# Autodesk Inventor assembly: DriverStation-ver2-1111-2021
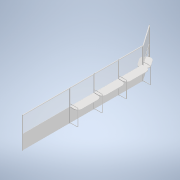
[picture p0: Inventor's stored thumbnail of the model, 180x180]
Saved by Autodesk Inventor 2021 (Build 250183000, 183)
## iProperties
Created: 2021-03-02
Part Number: DriverStation-ver2-1111-2021
Document SubType Name: Assembly
Designer: CMurray
Author: CMurray
## Documents named in this file (14)
- F:\PHRC CADD 2021\2021 Game Design Challenge\Player Station\Assemblies\DriverStation-ver2-1111-2021.iam
- F:\PHRC CADD 2021\2021 Game Design Challenge\Player Station\Parts\StationBase-ver1-1111-2021.ipt
- F:\PHRC CADD 2021\2021 Game Design Challenge\Player Station\Parts\StationDivider-ver1-1111-2021.iam
- F:\PHRC CADD 2021\2021 Game Design Challenge\Player Station\Parts\HPStationBase-ver1-1111-2021.ipt
- F:\PHRC CADD 2021\2021 Game Design Challenge\Player Station\Parts\StationDividerNoArm-ver1-1111-2021.iam
- F:\PHRC CADD 2021\2021 Game Design Challenge\Player Station\Parts\PSHalfWall-ver2-1111-2021.ipt
- F:\PHRC CADD 2021\2021 Game Design Challenge\Player Station\Parts\StationWindow-ver1-1111-2021.ipt
- F:\PHRC CADD 2021\2021 Game Design Challenge\Player Station\Parts\TopBar-ver1-1111-2021.ipt
- F:\PHRC CADD 2021\2021 Game Design Challenge\Player Station\Parts\TopBar-ver2-1111-2021.ipt
- F:\PHRC CADD 2021\2021 Game Design Challenge\Player Station\Parts\StationWindow-ver2-1111-2021.ipt
- F:\PHRC CADD 2021\2021 Game Design Challenge\Player Station\Parts\TopBar-ver3-1111-2021.ipt
- F:\PHRC CADD 2021\2021 Game Design Challenge\Player Station\Parts\StationWindow-ver3-1111-2021.ipt
- F:\PHRC CADD 2021\2021 Game Design Challenge\Player Station\Parts\Shelf-ver1-1111-2021.ipt
- F:\PHRC CADD 2021\2021 Game Design Challenge\Player Station\Parts\Shelf-ver2-1111-2021.ipt
## Components (26 placed, 13 different names)
1. StationBase-ver1-1111-2021:1 — Mate:1, Flush:1, Flush:2, Flush:3, Mate:2, Flush:4, Flush:7, Flush:8, Flush:11, Flush:12, Mate:21, Flush:34, Flush:40, Mate:30
2. StationDivider-ver1-1111-2021:1 [sub-assembly] — Mate:1, Flush:1, Flush:2, Mate:6, Mate:14, Flush:23, Flush:24, Mate:24, Mate:31
3. StationDivider-ver1-1111-2021:2 [sub-assembly] — Flush:3, Mate:2, Flush:4, Mate:4, Angle:2, Mate:15, Flush:25, Flush:26, Mate:22, Mate:33
4. StationBase-ver1-1111-2021:2 — Mate:4, Flush:7, Flush:8, Mate:9, Flush:16, Flush:17, Angle:3, Mate:19, Flush:33, Flush:41, Mate:32
5. StationBase-ver1-1111-2021:3 — Flush:11, Flush:12, Mate:6, Flush:19, Flush:20, Mate:23, Flush:35, Mate:28, Mate:29, Flush:39
6. StationDivider-ver1-1111-2021:4 [sub-assembly] — Mate:12, Flush:37, Mate:27
7. StationDivider-ver1-1111-2021:6 [sub-assembly] — Mate:9, Flush:16, Angle:2, Mate:10, Angle:4, Mate:16, Flush:27, Flush:28, Mate:20
8. HPStationBase-ver1-1111-2021:1 — Mate:10, Flush:17, Angle:3, Mate:11, Flush:18, Flush:29, Mate:17, Flush:30, Mate:34, Mate:35, Flush:42, Mate:36, Mate:37
9. StationDividerNoArm-ver1-1111-2021:1 [sub-assembly] — Mate:11, Angle:4, Flush:18
10. PSHalfWall-ver2-1111-2021:1 — Flush:19, Flush:20, Mate:12, Mate:13, Flush:21, Flush:22, Flush:36, Flush:38, Mate:26
11. StationDividerNoArm-ver1-1111-2021:2 [sub-assembly] — Mate:13, Flush:21, Flush:22, Mate:25
12. TopBar-ver1-1111-2021:1 — Mate:14, Flush:23, Flush:24
13. TopBar-ver1-1111-2021:2 — Mate:15, Flush:25, Flush:26
14. TopBar-ver1-1111-2021:3 — Mate:16, Flush:27, Flush:28
15. StationWindow-ver2-1111-2021:1 — Flush:29, Mate:17, Flush:30, Mate:18, Flush:31, Flush:32
16. TopBar-ver2-1111-2021:2 — Mate:18, Flush:31, Flush:32
17. StationWindow-ver1-1111-2021:1 — Mate:19, Flush:33, Mate:20
18. StationWindow-ver1-1111-2021:2 — Mate:21, Flush:34, Mate:22
19. StationWindow-ver1-1111-2021:3 — Mate:23, Flush:35, Mate:24
20. TopBar-ver3-1111-2021:1 — Mate:25, Flush:36, Flush:37
21. StationWindow-ver3-1111-2021:1 — Flush:38, Mate:26, Mate:27
22. Shelf-ver1-1111-2021:1 — Mate:28, Mate:29, Flush:39
23. Shelf-ver1-1111-2021:2 — Flush:40, Mate:30, Mate:31
24. Shelf-ver1-1111-2021:3 — Flush:41, Mate:32, Mate:33
25. Shelf-ver2-1111-2021:1 — Mate:34, Mate:35, Flush:42, Flush:43
26. Shelf-ver2-1111-2021:2 — Mate:36, Flush:43, Mate:37
## Relationships (75: Flush 38, Mate 34, Angle 3)
- Mate:1: StationBase-ver1-1111-2021:1 ↔ StationDivider-ver1-1111-2021:1
- Flush:1: StationBase-ver1-1111-2021:1 ↔ StationDivider-ver1-1111-2021:1
- Flush:2: StationBase-ver1-1111-2021:1 ↔ StationDivider-ver1-1111-2021:1
- Flush:3: StationBase-ver1-1111-2021:1 ↔ StationDivider-ver1-1111-2021:2
- Mate:2: StationBase-ver1-1111-2021:1 ↔ StationDivider-ver1-1111-2021:2
- Flush:4: StationBase-ver1-1111-2021:1 ↔ StationDivider-ver1-1111-2021:2
- Mate:4: StationDivider-ver1-1111-2021:2 ↔ StationBase-ver1-1111-2021:2
- Flush:7: StationBase-ver1-1111-2021:1 ↔ StationBase-ver1-1111-2021:2
- Flush:8: StationBase-ver1-1111-2021:1 ↔ StationBase-ver1-1111-2021:2
- [Mate]: StationBase-ver1-1111-2021:3 ↔ StationDivider-ver1-1111-2021:4
- [Flush]: StationBase-ver1-1111-2021:3 ↔ StationDivider-ver1-1111-2021:4
- [Flush]: StationBase-ver1-1111-2021:3 ↔ StationDivider-ver1-1111-2021:4
- Flush:11: StationBase-ver1-1111-2021:1 ↔ StationBase-ver1-1111-2021:3
- Flush:12: StationBase-ver1-1111-2021:1 ↔ StationBase-ver1-1111-2021:3
- Mate:6: StationDivider-ver1-1111-2021:1 ↔ StationBase-ver1-1111-2021:3
- Mate:9: StationBase-ver1-1111-2021:2 ↔ StationDivider-ver1-1111-2021:6
- Flush:16: StationBase-ver1-1111-2021:2 ↔ StationDivider-ver1-1111-2021:6
- Angle:2 (0 deg): StationDivider-ver1-1111-2021:2 ↔ StationDivider-ver1-1111-2021:6
- Mate:10: StationDivider-ver1-1111-2021:6 ↔ HPStationBase-ver1-1111-2021:1
- Flush:17: StationBase-ver1-1111-2021:2 ↔ HPStationBase-ver1-1111-2021:1
- Angle:3 (35 deg): StationBase-ver1-1111-2021:2 ↔ HPStationBase-ver1-1111-2021:1
- Mate:11: HPStationBase-ver1-1111-2021:1 ↔ StationDividerNoArm-ver1-1111-2021:1
- Angle:4 (0 deg): StationDivider-ver1-1111-2021:6 ↔ StationDividerNoArm-ver1-1111-2021:1
- Flush:18: HPStationBase-ver1-1111-2021:1 ↔ StationDividerNoArm-ver1-1111-2021:1
- Flush:19: StationBase-ver1-1111-2021:3 ↔ PSHalfWall-ver2-1111-2021:1
- Flush:20: StationBase-ver1-1111-2021:3 ↔ PSHalfWall-ver2-1111-2021:1
- Mate:12: StationDivider-ver1-1111-2021:4 ↔ PSHalfWall-ver2-1111-2021:1
- Mate:13: PSHalfWall-ver2-1111-2021:1 ↔ StationDividerNoArm-ver1-1111-2021:2
- Flush:21: PSHalfWall-ver2-1111-2021:1 ↔ StationDividerNoArm-ver1-1111-2021:2
- Flush:22: PSHalfWall-ver2-1111-2021:1 ↔ StationDividerNoArm-ver1-1111-2021:2
- Mate:14: StationDivider-ver1-1111-2021:1 ↔ TopBar-ver1-1111-2021:1
- Flush:23: StationDivider-ver1-1111-2021:1 ↔ TopBar-ver1-1111-2021:1
- Flush:24: StationDivider-ver1-1111-2021:1 ↔ TopBar-ver1-1111-2021:1
- Mate:15: StationDivider-ver1-1111-2021:2 ↔ TopBar-ver1-1111-2021:2
- Flush:25: StationDivider-ver1-1111-2021:2 ↔ TopBar-ver1-1111-2021:2
- Flush:26: StationDivider-ver1-1111-2021:2 ↔ TopBar-ver1-1111-2021:2
- Mate:16: StationDivider-ver1-1111-2021:6 ↔ TopBar-ver1-1111-2021:3
- Flush:27: StationDivider-ver1-1111-2021:6 ↔ TopBar-ver1-1111-2021:3
- Flush:28: StationDivider-ver1-1111-2021:6 ↔ TopBar-ver1-1111-2021:3
- Flush:29: HPStationBase-ver1-1111-2021:1 ↔ StationWindow-ver2-1111-2021:1
- Mate:17: HPStationBase-ver1-1111-2021:1 ↔ StationWindow-ver2-1111-2021:1
- Flush:30: HPStationBase-ver1-1111-2021:1 ↔ StationWindow-ver2-1111-2021:1
- Mate:18: StationWindow-ver2-1111-2021:1 ↔ TopBar-ver2-1111-2021:2
- Flush:31: StationWindow-ver2-1111-2021:1 ↔ TopBar-ver2-1111-2021:2
- Flush:32: StationWindow-ver2-1111-2021:1 ↔ TopBar-ver2-1111-2021:2
- Mate:19: StationBase-ver1-1111-2021:2 ↔ StationWindow-ver1-1111-2021:1
- Flush:33: StationBase-ver1-1111-2021:2 ↔ StationWindow-ver1-1111-2021:1
- Mate:20: StationDivider-ver1-1111-2021:6 ↔ StationWindow-ver1-1111-2021:1
- Mate:21: StationBase-ver1-1111-2021:1 ↔ StationWindow-ver1-1111-2021:2
- Flush:34: StationBase-ver1-1111-2021:1 ↔ StationWindow-ver1-1111-2021:2
- Mate:22: StationDivider-ver1-1111-2021:2 ↔ StationWindow-ver1-1111-2021:2
- Mate:23: StationBase-ver1-1111-2021:3 ↔ StationWindow-ver1-1111-2021:3
- Flush:35: StationBase-ver1-1111-2021:3 ↔ StationWindow-ver1-1111-2021:3
- Mate:24: StationDivider-ver1-1111-2021:1 ↔ StationWindow-ver1-1111-2021:3
- Mate:25: StationDividerNoArm-ver1-1111-2021:2 ↔ TopBar-ver3-1111-2021:1
- Flush:36: PSHalfWall-ver2-1111-2021:1 ↔ TopBar-ver3-1111-2021:1
- Flush:37: StationDivider-ver1-1111-2021:4 ↔ TopBar-ver3-1111-2021:1
- Flush:38: PSHalfWall-ver2-1111-2021:1 ↔ StationWindow-ver3-1111-2021:1
- Mate:26: PSHalfWall-ver2-1111-2021:1 ↔ StationWindow-ver3-1111-2021:1
- Mate:27: StationDivider-ver1-1111-2021:4 ↔ StationWindow-ver3-1111-2021:1
- Mate:28: StationBase-ver1-1111-2021:3 ↔ Shelf-ver1-1111-2021:1
- Mate:29: StationBase-ver1-1111-2021:3 ↔ Shelf-ver1-1111-2021:1
- Flush:39: StationBase-ver1-1111-2021:3 ↔ Shelf-ver1-1111-2021:1
- Flush:40: StationBase-ver1-1111-2021:1 ↔ Shelf-ver1-1111-2021:2
- Mate:30: StationBase-ver1-1111-2021:1 ↔ Shelf-ver1-1111-2021:2
- Mate:31: StationDivider-ver1-1111-2021:1 ↔ Shelf-ver1-1111-2021:2
- Flush:41: StationBase-ver1-1111-2021:2 ↔ Shelf-ver1-1111-2021:3
- Mate:32: StationBase-ver1-1111-2021:2 ↔ Shelf-ver1-1111-2021:3
- Mate:33: StationDivider-ver1-1111-2021:2 ↔ Shelf-ver1-1111-2021:3
- Mate:34: HPStationBase-ver1-1111-2021:1 ↔ Shelf-ver2-1111-2021:1
- Mate:35: HPStationBase-ver1-1111-2021:1 ↔ Shelf-ver2-1111-2021:1
- Flush:42: HPStationBase-ver1-1111-2021:1 ↔ Shelf-ver2-1111-2021:1
- Mate:36: HPStationBase-ver1-1111-2021:1 ↔ Shelf-ver2-1111-2021:2
- Flush:43: Shelf-ver2-1111-2021:1 ↔ Shelf-ver2-1111-2021:2
- Mate:37: HPStationBase-ver1-1111-2021:1 ↔ Shelf-ver2-1111-2021:2
## Named parameters: d12_d0 = 0 mm, d13_d1 = 0 mm, d14_d2 = 0 mm
